# Autodesk Inventor assembly: Assembly
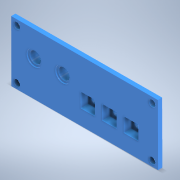
[picture p0: Inventor's stored thumbnail of the model, 180x180]
Saved by Autodesk Inventor 2022.2 (Build 262287000, 287)
## iProperties
Created: 2022-01-15
Part Number: Assembly
Document SubType Name: Assembly
Designer: siwat
Author: siwat
## Documents named in this file (19)
- D:\Git\osu-cbt\CAD\Assembly.iam
- D:\Git\osu-cbt\CAD\LM2596 DC to DC Buck Converter 3 A.ipt
- D:\Git\osu-cbt\CAD\due\ARDUINO DUE.iam
- D:\Git\osu-cbt\CAD\3V210-08NC, 2 POSITION, 3 WAY SOLENOID VALVE\3V210-08NC, 2 POSITION, 3 WAY SOLENOID VALVE.iam
- D:\Git\osu-cbt\CAD\S-60-12.ipt
- D:\Git\osu-cbt\CAD\Base.ipt
- D:\Git\osu-cbt\CAD\RelayTray.ipt
- D:\Git\osu-cbt\CAD\CoverPSU.ipt
- D:\Git\osu-cbt\CAD\2PH63091A Parts\Relay - 2 Channel - 2PH63091A - Montaj.iam
- D:\Git\osu-cbt\CAD\Lid.ipt
- D:\Git\osu-cbt\CAD\Assembly\AIP\Tube and Pipe\Assembly.Tube and Pipe Runs.iam
- D:\Git\osu-cbt\CAD\Assembly\AIP\Cable and Harness\Assembly.Harness1.iam
- D:\Git\osu-cbt\CAD\InterfacePlate.ipt
- D:\Git\osu-cbt\CAD\5mm LED.ipt
- D:\Git\osu-cbt\CAD\LED_YELLOW.ipt
- D:\Git\osu-cbt\CAD\Tactal Switch -Thru 6x 6x10.ipt
- D:\Git\osu-cbt\CAD\Releases\Prototype 1\BaseTextWhite.ipt
- D:\Git\osu-cbt\CAD\Releases\Prototype 1\BaseTextYellow.ipt
- D:\Git\osu-cbt\CAD\InterfacePlateTextOrange.ipt
## Components (21 placed, 18 different names)
1. LM2596 DC to DC Buck Converter 3 A:1
2. ARDUINO DUE:1 [sub-assembly]
3. 3V210-08NC, 2 POSITION, 3 WAY SOLENOID VALVE:1 [sub-assembly]
4. S-60-12:1
5. Base:1 — Flush:1, Flush:2, Flush:3, Flush:4, Flush:5, Flush:6, Flush:9, Flush:10, Flush:11, Flush:12, Flush:13, Flush:14, Flush:15, Flush:16, Flush:17, Flush:18, Insert:1, Flush:19, Flush:20
6. RelayTray:1 — Flush:1, Flush:2
7. CoverPSU:1 — Flush:3, Flush:4, Insert:1
8. Relay - 2 Channel - 2PH63091A - Montaj:1 [sub-assembly]
9. Lid:1 — Flush:5, Flush:6
10. Tube & Pipe Runs [sub-assembly]
11. Harness1 [sub-assembly]
12. 3V210-08NC, 2 POSITION, 3 WAY SOLENOID VALVE:2 [sub-assembly]
13. InterfacePlate:1 — Flush:21, Flush:22
14. 5mm LED:1
15. LED_YELLOW:1
16. Tactal Switch -Thru 6x 6x10:1
17. Tactal Switch -Thru 6x 6x10:2
18. Tactal Switch -Thru 6x 6x10:3
19. BaseTextWhite:1 — Flush:9, Flush:10, Flush:11, Flush:12, Flush:13, Flush:20
20. BaseTextYellow:1 — Flush:14, Flush:15, Flush:16, Flush:17, Flush:18, Flush:19
21. InterfacePlateTextOrange:1 — Flush:21, Flush:22
## Relationships (21: Flush 20, Insert 1)
- Flush:1: Base:1 ↔ RelayTray:1
- Flush:2: Base:1 ↔ RelayTray:1
- Flush:3: Base:1 ↔ CoverPSU:1
- Flush:4: Base:1 ↔ CoverPSU:1
- Flush:5: Base:1 ↔ Lid:1
- Flush:6: Base:1 ↔ Lid:1
- Flush:9: Base:1 ↔ BaseTextWhite:1
- Flush:10: Base:1 ↔ BaseTextWhite:1
- Flush:11: Base:1 ↔ BaseTextWhite:1
- Flush:12: Base:1 ↔ BaseTextWhite:1
- Flush:13: Base:1 ↔ BaseTextWhite:1
- Flush:14: Base:1 ↔ BaseTextYellow:1
- Flush:15: Base:1 ↔ BaseTextYellow:1
- Flush:16: Base:1 ↔ BaseTextYellow:1
- Flush:17: Base:1 ↔ BaseTextYellow:1
- Flush:18: Base:1 ↔ BaseTextYellow:1
- Insert:1: Base:1 ↔ CoverPSU:1
- Flush:19: Base:1 ↔ BaseTextYellow:1
- Flush:20: Base:1 ↔ BaseTextWhite:1
- Flush:21: InterfacePlate:1 ↔ InterfacePlateTextOrange:1
- Flush:22: InterfacePlate:1 ↔ InterfacePlateTextOrange:1
